# Autodesk Inventor assembly: Ensamblaje Caja para Electrónica
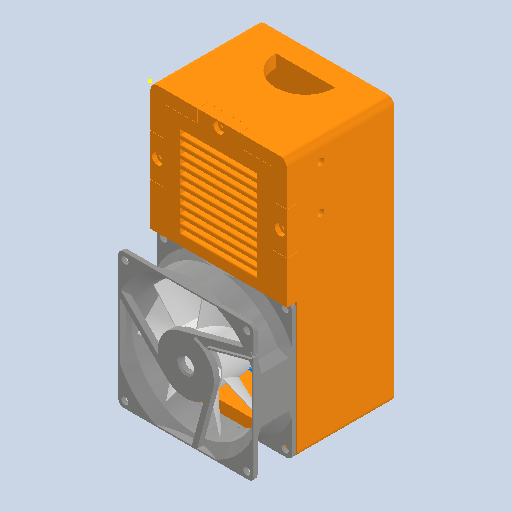
[picture p0: Inventor's stored thumbnail of the model, 512x512]
Saved by Autodesk Inventor 2026 (Build 300175050, 175E)
## iProperties
Created: 2026-02-11
Part Number: Ensamblaje Caja para Electrónica
Document SubType Name: Assembly
Designer: bello
Author: bello
## Documents named in this file (6)
- A:\Federico Bellomi\UNLZ\5. Quinto Año\Proyecto Final\Ensamblaje\Eje Z\Ensamblaje Caja para Electrónica.iam
- A:\Federico Bellomi\UNLZ\5. Quinto Año\Proyecto Final\Ensamblaje\Eje Z\Caja para Electrónica.ipt
- A:\Federico Bellomi\UNLZ\5. Quinto Año\Proyecto Final\Ensamblaje\Eje Z\RepRap\RepRap\RepRap.ipt
- A:\Federico Bellomi\UNLZ\5. Quinto Año\Proyecto Final\Ensamblaje\Eje Z\TCA9548A\TCA9548A.ipt
- A:\Federico Bellomi\UNLZ\5. Quinto Año\Proyecto Final\Ensamblaje\Eje Z\80MM_FAN\80MM_FAN\80MM_FAN.ipt
- A:\Federico Bellomi\UNLZ\5. Quinto Año\Proyecto Final\Ensamblaje\Eje Z\Tapa - Caja para Electrónica.ipt
## Components (5 placed, 5 different names)
1. Caja para Electrónica:1 — Coincidencia:1, Coincidencia:2, Coincidencia:3, Coincidencia:4, Coincidencia:5, Nivelación:1, Nivelación:2, Coincidencia:6, Coincidencia:7, Coincidencia:8
2. RepRap:1 — Coincidencia:1, Coincidencia:2
3. TCA9548A:1 — Coincidencia:3, Coincidencia:4
4. 80MM_FAN:1 — Coincidencia:5, Nivelación:1, Nivelación:2
5. Tapa - Caja para Electrónica:1 — Coincidencia:6, Coincidencia:7, Coincidencia:8
## Relationships (10: Mate 8, Flush 2)
- Coincidencia:1 [Mate]: Caja para Electrónica:1 ↔ RepRap:1
- Coincidencia:2 [Mate] (0.5 mm): Caja para Electrónica:1 ↔ RepRap:1
- Coincidencia:3 [Mate]: Caja para Electrónica:1 ↔ TCA9548A:1
- Coincidencia:4 [Mate] (1.5 mm): Caja para Electrónica:1 ↔ TCA9548A:1
- Coincidencia:5 [Mate]: Caja para Electrónica:1 ↔ 80MM_FAN:1
- Nivelación:1 [Flush]: Caja para Electrónica:1 ↔ 80MM_FAN:1
- Nivelación:2 [Flush]: Caja para Electrónica:1 ↔ 80MM_FAN:1
- Coincidencia:6 [Mate]: Caja para Electrónica:1 ↔ Tapa - Caja para Electrónica:1
- Coincidencia:7 [Mate]: Caja para Electrónica:1 ↔ Tapa - Caja para Electrónica:1
- Coincidencia:8 [Mate]: Caja para Electrónica:1 ↔ Tapa - Caja para Electrónica:1
